# Autodesk Inventor assembly: enc - SidePanel Oben V2 - Assembly
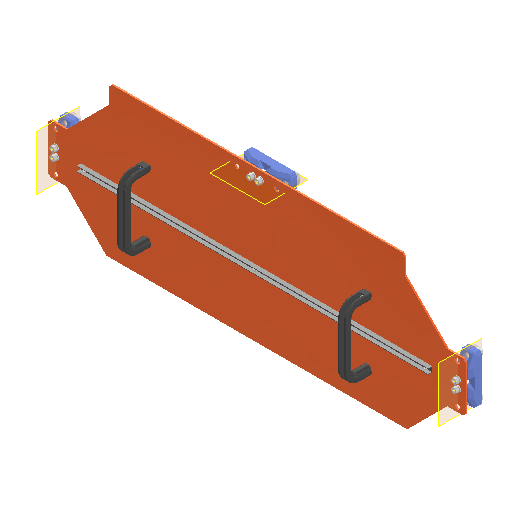
[picture p0: Inventor's stored thumbnail of the model, 512x512]
Saved by Autodesk Inventor 2023.2 (Build 272271000, 271)
## iProperties
Created: 2023-12-14
Part Number: enc - SidePanel Oben V2 - Assembly
Document SubType Name: Assembly
Designer: Nils Bade
Author: Nils Bade
## Documents named in this file (7)
- C:\Users\nilsb\Documents\Inventor\Projektarbeit-Bade\Enclosure\enc - SidePanel Oben V2 - Assembly.iam
- C:\Users\nilsb\Documents\Inventor\Projektarbeit-Bade\Enclosure\enc - SidePanel Oben V2.ipt
- C:\Users\nilsb\Documents\Inventor\Projektarbeit-Bade\Enclosure\Magnet PanelFrame Straight connected.iam
- C:\Users\nilsb\Documents\Inventor\Projektarbeit-Bade\Enclosure\U-Profil PanelSupport 10x8x660mm.ipt
- C:\Users\nilsb\Documents\Inventor\Projektarbeit-Bade\Schrauben\Cap Head Screw M4x8 - DIN912.ipt
- C:\Users\nilsb\Documents\Inventor\Projektarbeit-Bade\RatRig_Standards\Hex Nut - M4 DIN934.ipt
- C:\Users\nilsb\Documents\Inventor\Projektarbeit-Bade\Enclosure\item_Handgriff_PA120_Assembly.iam
## Components (13 placed, 6 different names)
1. Magnet PanelFrame Straight connected:1 [sub-assembly] — Passend:4, Passend:5, Passend:6
2. Magnet PanelFrame Straight connected:2 [sub-assembly] — Passend:7, Passend:8, Passend:9
3. Magnet PanelFrame Straight connected:3 [sub-assembly] — Passend:1, Passend:2, Passend:3
4. item_Handgriff_120er:2 [sub-assembly] — Passend:25, Passend:28, Passend:29
5. item_Handgriff_120er:1 [sub-assembly] — Passend:26, Passend:27, Passend:30
6. Hex Nut - M4 DIN934:3 — Passend:21, Passend:24
7. Hex Nut - M4 DIN934:2 — Passend:20, Passend:23
8. Hex Nut - M4 DIN934:1 — Passend:19, Passend:22
9. Cap Head Screw M4x8 - DIN912:3 — Passend:15, Passend:18, Passend:19
10. Cap Head Screw M4x8 - DIN912:2 — Passend:14, Passend:17, Passend:20
11. Cap Head Screw M4x8 - DIN912:1 — Passend:13, Passend:16, Passend:21
12. U-Profil PanelSupport 10x8x265mm:1 — Passend:10, Passend:11, Passend:12, Passend:16, Passend:17, Passend:18
13. enc - SidePanel Oben V2 - 333x795:1 — Passend:1, Passend:2, Passend:3, Passend:4, Passend:5, Passend:6, Passend:7, Passend:8, Passend:9, Passend:10, Passend:11, Passend:12, Passend:13, Passend:14, Passend:15, Passend:22, Passend:23, Passend:24, Passend:25, Passend:26, Passend:27, Passend:28, Passend:29, Passend:30
## Relationships (30: Mate 30)
- Passend:1 [Mate]: Magnet PanelFrame Straight connected:3 ↔ enc - SidePanel Oben V2 - 333x795:1
- Passend:2 [Mate]: Magnet PanelFrame Straight connected:3 ↔ enc - SidePanel Oben V2 - 333x795:1
- Passend:3 [Mate]: Magnet PanelFrame Straight connected:3 ↔ enc - SidePanel Oben V2 - 333x795:1
- Passend:4 [Mate]: Magnet PanelFrame Straight connected:1 ↔ enc - SidePanel Oben V2 - 333x795:1
- Passend:5 [Mate]: Magnet PanelFrame Straight connected:1 ↔ enc - SidePanel Oben V2 - 333x795:1
- Passend:6 [Mate]: Magnet PanelFrame Straight connected:1 ↔ enc - SidePanel Oben V2 - 333x795:1
- Passend:7 [Mate]: Magnet PanelFrame Straight connected:2 ↔ enc - SidePanel Oben V2 - 333x795:1
- Passend:8 [Mate]: Magnet PanelFrame Straight connected:2 ↔ enc - SidePanel Oben V2 - 333x795:1
- Passend:9 [Mate]: Magnet PanelFrame Straight connected:2 ↔ enc - SidePanel Oben V2 - 333x795:1
- Passend:10 [Mate]: U-Profil PanelSupport 10x8x265mm:1 ↔ enc - SidePanel Oben V2 - 333x795:1
- Passend:11 [Mate]: U-Profil PanelSupport 10x8x265mm:1 ↔ enc - SidePanel Oben V2 - 333x795:1
- Passend:12 [Mate]: U-Profil PanelSupport 10x8x265mm:1 ↔ enc - SidePanel Oben V2 - 333x795:1
- Passend:13 [Mate]: Cap Head Screw M4x8 - DIN912:1 ↔ enc - SidePanel Oben V2 - 333x795:1
- Passend:14 [Mate]: Cap Head Screw M4x8 - DIN912:2 ↔ enc - SidePanel Oben V2 - 333x795:1
- Passend:15 [Mate]: Cap Head Screw M4x8 - DIN912:3 ↔ enc - SidePanel Oben V2 - 333x795:1
- Passend:16 [Mate]: Cap Head Screw M4x8 - DIN912:1 ↔ U-Profil PanelSupport 10x8x265mm:1
- Passend:17 [Mate]: Cap Head Screw M4x8 - DIN912:2 ↔ U-Profil PanelSupport 10x8x265mm:1
- Passend:18 [Mate]: Cap Head Screw M4x8 - DIN912:3 ↔ U-Profil PanelSupport 10x8x265mm:1
- Passend:19 [Mate]: Hex Nut - M4 DIN934:1 ↔ Cap Head Screw M4x8 - DIN912:3
- Passend:20 [Mate]: Hex Nut - M4 DIN934:2 ↔ Cap Head Screw M4x8 - DIN912:2
- Passend:21 [Mate]: Hex Nut - M4 DIN934:3 ↔ Cap Head Screw M4x8 - DIN912:1
- Passend:22 [Mate]: Hex Nut - M4 DIN934:1 ↔ enc - SidePanel Oben V2 - 333x795:1
- Passend:23 [Mate]: Hex Nut - M4 DIN934:2 ↔ enc - SidePanel Oben V2 - 333x795:1
- Passend:24 [Mate]: Hex Nut - M4 DIN934:3 ↔ enc - SidePanel Oben V2 - 333x795:1
- Passend:25 [Mate]: item_Handgriff_120er:2 ↔ enc - SidePanel Oben V2 - 333x795:1
- Passend:26 [Mate]: item_Handgriff_120er:1 ↔ enc - SidePanel Oben V2 - 333x795:1
- Passend:27 [Mate]: item_Handgriff_120er:1 ↔ enc - SidePanel Oben V2 - 333x795:1
- Passend:28 [Mate]: item_Handgriff_120er:2 ↔ enc - SidePanel Oben V2 - 333x795:1
- Passend:29 [Mate]: item_Handgriff_120er:2 ↔ enc - SidePanel Oben V2 - 333x795:1
- Passend:30 [Mate]: item_Handgriff_120er:1 ↔ enc - SidePanel Oben V2 - 333x795:1
